# Autodesk Inventor assembly: House_Assembly
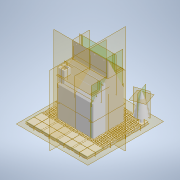
[picture p0: Inventor's stored thumbnail of the model, 180x180]
Saved by Autodesk Inventor 2022.4 (Build 264492010, 492A)
## iProperties
Created: 2025-02-20
Part Number: House_Assembly
Document SubType Name: Assembly
Designer: jan-m
Author: jan-m
## Documents named in this file (20)
- C:\School\Masterproef\3D Modellen\House_Assembly_Depth_Tracking.iam
- C:\School\Masterproef\3D Modellen\Tile.ipt
- C:\School\Masterproef\3D Modellen\Tile_Connector.ipt
- C:\School\Masterproef\3D Modellen\Wall.ipt
- C:\School\Masterproef\3D Modellen\Roof_Wall_Small_Left.ipt
- C:\School\Masterproef\3D Modellen\Roof_Wall_Small_Right.ipt
- C:\School\Masterproef\3D Modellen\Roof_Wall_Large_Left.ipt
- C:\School\Masterproef\3D Modellen\Roof_Wall_Large_Right.ipt
- C:\School\Masterproef\3D Modellen\Roof_Small.ipt
- C:\School\Masterproef\3D Modellen\Roof_Large.ipt
- C:\School\Masterproef\3D Modellen\Hanging_Wall.ipt
- C:\School\Masterproef\3D Modellen\1x1_Piece.ipt
- C:\School\Masterproef\3D Modellen\Tile_Cover.ipt
- C:\School\Masterproef\3D Modellen\Tree_Leaves.ipt
- C:\School\Masterproef\3D Modellen\Tree_Trunk.ipt
- C:\School\Masterproef\3D Modellen\Chimney.ipt
- C:\School\Masterproef\3D Modellen\Pin.ipt
- C:\School\Masterproef\3D Modellen\Rail_Clip_Left.ipt
- C:\School\Masterproef\3D Modellen\Rail_Clip_Right.ipt
- C:\School\Masterproef\3D Modellen\Roof_Pin_Clip.ipt
## Components (251 placed, 19 different names)
1. Wall:1 — Mate:10, Mate:11, Mate:12, Mate:40, Mate:46, Mate:59
2. Wall:2 — Mate:13, Mate:14, Mate:15, Mate:27, Mate:28, Mate:30, Mate:31, Mate:60, Mate:64, Mate:72
3. Wall:3 — Mate:19, Mate:20, Mate:21, Mate:37, Mate:42, Mate:58
4. Wall:4 — Mate:16, Mate:17, Mate:18, Mate:23, Mate:25, Mate:33, Mate:34, Mate:63, Mate:65
5. Roof_Wall_Small_Left:2 — Mate:23, Mate:25, Mate:65, Mate:80, Mate:81, Flush:6, Mate:102, Flush:12, Angle:1
6. Roof_Wall_Small_Right:2 — Mate:27, Mate:28, Mate:64, Mate:72, Mate:101, Mate:103, Flush:13, Angle:2
7. Roof_Wall_Large_Left:1 — Mate:30, Mate:31, Mate:60, Mate:106, Flush:16, Angle:5, Mate:107, Flush:17, Angle:6
8. Roof_Wall_Large_Right:1 — Mate:33, Mate:34, Mate:63, Mate:98, Mate:104, Flush:14, Angle:3, Mate:105, Flush:15, Angle:4
9. Roof_Small:1 — Mate:37, Mate:42, Mate:58, Mate:96, Mate:97, Mate:99, Mate:100
10. Roof_Large:1 — Mate:40, Mate:43, Mate:44, Mate:46, Mate:59, Flush:7
11. Hanging_Wall:1 — Mate:43, Mate:44, Flush:7
12. Tree_Leaves:1 — Mate:73, Mate:74
13. Tree_Trunk:1 — Mate:73, Mate:74, Mate:75, Mate:76, Mate:77
14. Chimney:1 — Mate:78, Mate:79, Mate:81, Flush:6
15. Pin:1 — Mate:78, Mate:79, Mate:80
16. Rail_Clip_Left:1 — Mate:96, Mate:97, Mate:98
17. Rail_Clip_Right:1 — Mate:99, Mate:100, Mate:101
18. Roof_Pin_Clip:1 — Mate:105, Flush:15, Angle:4
19. Roof_Pin_Clip:2 — Mate:106, Flush:16, Angle:5
20. Roof_Pin_Clip:3 — Mate:104, Flush:14, Angle:3
21. Roof_Pin_Clip:4 — Mate:102, Flush:12, Angle:1
22. Roof_Pin_Clip:5 — Mate:107, Flush:17, Angle:6
23. Roof_Pin_Clip:6 — Mate:103, Flush:13, Angle:2
24. Tile_Connector:2 — Mate:6, Mate:7
25. Tile:1 — Mate:2, Mate:5, Mate:6, Mate:7, Mate:16, Mate:91, Mate:92
26. Tile_Connector:1 — Mate:2, Mate:5
27. Tile_Connector:3
28. Tile:2 — Mate:10, Mate:12
29. Tile_Connector:4
30. Tile_Connector:5
31. Tile:3 — Mate:11
32. Tile_Connector:6
33. Tile_Connector:7
34. Tile:4 — Mate:13, Mate:75, Mate:76, Mate:77, Mate:94, Mate:95, Flush:11
35. Tile_Connector:8
36. Tile_Connector:9
37. Tile:5
38. Tile_Connector:10
39. Tile_Connector:11
40. Tile:6
41. Tile_Connector:12
42. Tile_Connector:13
43. Tile:7 — Mate:82, Flush:9
44. Tile_Connector:14
45. Tile_Connector:15
46. Tile:8 — Mate:15
47. Tile_Connector:16
48. Tile_Connector:17
49. Tile:9 — Mate:17, Mate:18, Mate:83, Mate:84, Flush:10, Mate:85, Mate:86
50. Tile_Connector:18
51. Tile_Connector:19
52. Tile:10 — Mate:19, Mate:21
53. Tile_Connector:20
54. Tile_Connector:21
55. Tile:11 — Mate:20
56. Tile_Connector:22
57. Tile_Connector:23
58. Tile:12 — Mate:14, Mate:88, Mate:89
59. Tile_Connector:24
60. Tile_Connector:25
61. Tile:13 — Mate:57, Mate:61, Mate:62
62. Tile_Connector:26
63. Tile_Connector:27
64. Tile:14
65. Tile_Connector:28
66. Tile_Connector:29
67. Tile:15
68. Tile_Connector:30
69. Tile_Connector:31
70. Tile:16
71. Tile_Connector:32
72. Tile_Cover:1 — Mate:57, Mate:61, Mate:62
73. Tile_Cover:2
74. Tile_Cover:3
75. Tile_Cover:4
76. 1x1_Piece:147 — Mate:83, Mate:84, Flush:10
77. 1x1_Piece:155
78. 1x1_Piece:156
79. 1x1_Piece:157 — Mate:87
80. 1x1_Piece:158
81. 1x1_Piece:159
82. 1x1_Piece:160
83. 1x1_Piece:161
84. 1x1_Piece:162
85. 1x1_Piece:163
86. 1x1_Piece:164
87. 1x1_Piece:165
88. 1x1_Piece:166
89. 1x1_Piece:167
90. 1x1_Piece:168
91. 1x1_Piece:169
92. 1x1_Piece:170
93. 1x1_Piece:171
94. 1x1_Piece:172
95. 1x1_Piece:173
96. 1x1_Piece:174
97. 1x1_Piece:175
98. 1x1_Piece:176
99. 1x1_Piece:177
100. 1x1_Piece:178
101. 1x1_Piece:179
102. 1x1_Piece:180
103. 1x1_Piece:181
104. 1x1_Piece:182
105. 1x1_Piece:183
106. 1x1_Piece:184
107. 1x1_Piece:185
108. 1x1_Piece:186
109. 1x1_Piece:187
110. 1x1_Piece:188
111. 1x1_Piece:189
112. 1x1_Piece:190
113. 1x1_Piece:191
114. 1x1_Piece:192
115. 1x1_Piece:193
116. 1x1_Piece:194
117. 1x1_Piece:195
118. 1x1_Piece:196
119. 1x1_Piece:197
120. 1x1_Piece:198
121. 1x1_Piece:199
122. 1x1_Piece:200
123. 1x1_Piece:201 — Mate:93
124. 1x1_Piece:202
125. 1x1_Piece:203
126. 1x1_Piece:204
127. 1x1_Piece:205
128. 1x1_Piece:206
129. 1x1_Piece:207
130. 1x1_Piece:208
131. 1x1_Piece:209
132. 1x1_Piece:210
133. 1x1_Piece:211
134. 1x1_Piece:212
135. 1x1_Piece:213
136. 1x1_Piece:146 — Mate:85, Mate:86, Mate:87
137. 1x1_Piece:214
138. 1x1_Piece:215
139. 1x1_Piece:216
140. 1x1_Piece:217
141. 1x1_Piece:218
142. 1x1_Piece:219
143. 1x1_Piece:220
144. 1x1_Piece:221
145. 1x1_Piece:222
146. 1x1_Piece:223
147. 1x1_Piece:224 — Mate:90
148. 1x1_Piece:151 — Mate:88, Mate:89, Mate:90
149. 1x1_Piece:225
150. 1x1_Piece:226
151. 1x1_Piece:227
152. 1x1_Piece:228
153. 1x1_Piece:229
154. 1x1_Piece:230
155. 1x1_Piece:231
156. 1x1_Piece:232
157. 1x1_Piece:233
158. 1x1_Piece:234
159. 1x1_Piece:235
160. 1x1_Piece:236
161. 1x1_Piece:237
162. 1x1_Piece:238
163. 1x1_Piece:239
164. 1x1_Piece:240
165. 1x1_Piece:241
166. 1x1_Piece:242
167. 1x1_Piece:243
168. 1x1_Piece:244
169. 1x1_Piece:245
170. 1x1_Piece:246
171. 1x1_Piece:247
172. 1x1_Piece:248
173. 1x1_Piece:249
174. 1x1_Piece:250
175. 1x1_Piece:251
176. 1x1_Piece:252
177. 1x1_Piece:253
178. 1x1_Piece:254
179. 1x1_Piece:255
180. 1x1_Piece:256
181. 1x1_Piece:257
182. 1x1_Piece:258
183. 1x1_Piece:259
184. 1x1_Piece:260
185. 1x1_Piece:261
186. 1x1_Piece:262
187. 1x1_Piece:263
188. 1x1_Piece:264
189. 1x1_Piece:265
190. 1x1_Piece:266
191. 1x1_Piece:267
192. 1x1_Piece:268
193. 1x1_Piece:269
194. 1x1_Piece:270
195. 1x1_Piece:271
196. 1x1_Piece:272
197. 1x1_Piece:273
198. 1x1_Piece:274
199. 1x1_Piece:275
200. 1x1_Piece:145 — Mate:91, Mate:92, Mate:93
201. 1x1_Piece:276
202. 1x1_Piece:277
203. 1x1_Piece:278
204. 1x1_Piece:279
205. 1x1_Piece:280
206. 1x1_Piece:281
207. 1x1_Piece:282
208. 1x1_Piece:283
209. 1x1_Piece:284
210. 1x1_Piece:285
211. 1x1_Piece:286
212. 1x1_Piece:287
213. 1x1_Piece:288
214. 1x1_Piece:289
215. 1x1_Piece:290
216. 1x1_Piece:291
217. 1x1_Piece:292
218. 1x1_Piece:293
219. 1x1_Piece:294
220. 1x1_Piece:295
221. 1x1_Piece:296
222. 1x1_Piece:297
223. 1x1_Piece:298
224. 1x1_Piece:299
225. 1x1_Piece:300
226. 1x1_Piece:301
227. 1x1_Piece:302
228. 1x1_Piece:303
229. 1x1_Piece:304
230. 1x1_Piece:305
231. 1x1_Piece:306
232. 1x1_Piece:307
233. 1x1_Piece:308
234. 1x1_Piece:309
235. 1x1_Piece:310
236. 1x1_Piece:311
237. 1x1_Piece:312
238. 1x1_Piece:313
239. 1x1_Piece:314
240. 1x1_Piece:315
241. 1x1_Piece:316
242. 1x1_Piece:317
243. 1x1_Piece:318
244. 1x1_Piece:319
245. 1x1_Piece:320
246. 1x1_Piece:321
247. 1x1_Piece:322
248. 1x1_Piece:148 — Mate:94, Mate:95, Flush:11
249. 1x1_Piece:323
250. 1x1_Piece:324
251. 1x1_Piece:325
## Component patterns: (16 elements, first: Tile_Connector:2 + Tile:1 + Tile_Connector:1), (4 elements, first: Tile_Cover:1), (60 elements, first: 1x1_Piece:147), (12 elements, first: 1x1_Piece:146), (52 elements, first: 1x1_Piece:151), (48 elements, first: 1x1_Piece:145), (4 elements, first: 1x1_Piece:148)
## Relationships (92: Mate 75, Flush 11, Angle 6)
- Mate:2: Tile:1 ↔ Tile_Connector:1
- Mate:5: Tile:1 ↔ Tile_Connector:1
- Mate:6: Tile_Connector:2 ↔ Tile:1
- Mate:7: Tile_Connector:2 ↔ Tile:1
- Mate:10: Wall:1 ↔ Tile:2
- Mate:11: Wall:1 ↔ Tile:3
- Mate:12: Wall:1 ↔ Tile:2
- Mate:13: Wall:2 ↔ Tile:4
- Mate:14: Wall:2 ↔ Tile:12
- Mate:15: Wall:2 ↔ Tile:8
- Mate:16: Wall:4 ↔ Tile:1
- Mate:17: Wall:4 ↔ Tile:9
- Mate:18: Wall:4 ↔ Tile:9
- Mate:19: Wall:3 ↔ Tile:10
- Mate:20: Wall:3 ↔ Tile:11
- Mate:21: Wall:3 ↔ Tile:10
- Mate:23: Wall:4 ↔ Roof_Wall_Small_Left:2
- Mate:25: Wall:4 ↔ Roof_Wall_Small_Left:2
- Mate:27: Wall:2 ↔ Roof_Wall_Small_Right:2
- Mate:28: Wall:2 ↔ Roof_Wall_Small_Right:2
- Mate:30: Wall:2 ↔ Roof_Wall_Large_Left:1
- Mate:31: Wall:2 ↔ Roof_Wall_Large_Left:1
- Mate:33: Wall:4 ↔ Roof_Wall_Large_Right:1
- Mate:34: Wall:4 ↔ Roof_Wall_Large_Right:1
- Mate:37: Wall:3 ↔ Roof_Small:1
- Mate:40: Wall:1 ↔ Roof_Large:1
- Mate:42: Wall:3 ↔ Roof_Small:1
- Mate:43: Roof_Large:1 ↔ Hanging_Wall:1
- Mate:44: Roof_Large:1 ↔ Hanging_Wall:1
- Mate:46: Wall:1 ↔ Roof_Large:1
- Mate:57: Tile:13 ↔ Tile_Cover:1
- Mate:58: Wall:3 ↔ Roof_Small:1
- Mate:59: Wall:1 ↔ Roof_Large:1
- Mate:60: Wall:2 ↔ Roof_Wall_Large_Left:1
- Mate:61: Tile:13 ↔ Tile_Cover:1
- Mate:62: Tile:13 ↔ Tile_Cover:1
- Mate:63: Wall:4 ↔ Roof_Wall_Large_Right:1
- Mate:64: Wall:2 ↔ Roof_Wall_Small_Right:2
- Mate:65: Wall:4 ↔ Roof_Wall_Small_Left:2
- Mate:72: Wall:2 ↔ Roof_Wall_Small_Right:2
- Mate:73: Tree_Leaves:1 ↔ Tree_Trunk:1
- Mate:74: Tree_Leaves:1 ↔ Tree_Trunk:1
- Mate:75: Tree_Trunk:1 ↔ Tile:4
- Mate:76: Tree_Trunk:1 ↔ Tile:4
- Mate:77: Tree_Trunk:1 ↔ Tile:4
- Mate:78: Chimney:1 ↔ Pin:1
- Mate:79: Chimney:1 ↔ Pin:1
- Mate:80: Roof_Wall_Small_Left:2 ↔ Pin:1
- Mate:81: Roof_Wall_Small_Left:2 ↔ Chimney:1
- Flush:6: Roof_Wall_Small_Left:2 ↔ Chimney:1
- Flush:7: Roof_Large:1 ↔ Hanging_Wall:1
- Mate:82: Tile:7
- Flush:9: Tile:7
- Mate:83: Tile:9 ↔ 1x1_Piece:147
- Mate:84: Tile:9 ↔ 1x1_Piece:147
- Flush:10: Tile:9 ↔ 1x1_Piece:147
- Mate:85: Tile:9 ↔ 1x1_Piece:146
- Mate:86: Tile:9 ↔ 1x1_Piece:146
- Mate:87: 1x1_Piece:157 ↔ 1x1_Piece:146
- Mate:88: Tile:12 ↔ 1x1_Piece:151
- Mate:89: Tile:12 ↔ 1x1_Piece:151
- Mate:90: 1x1_Piece:224 ↔ 1x1_Piece:151
- Mate:91: Tile:1 ↔ 1x1_Piece:145
- Mate:92: Tile:1 ↔ 1x1_Piece:145
- Mate:93: 1x1_Piece:201 ↔ 1x1_Piece:145
- Mate:94: Tile:4 ↔ 1x1_Piece:148
- Mate:95: Tile:4 ↔ 1x1_Piece:148
- Flush:11: Tile:4 ↔ 1x1_Piece:148
- Mate:96: Roof_Small:1 ↔ Rail_Clip_Left:1
- Mate:97: Roof_Small:1 ↔ Rail_Clip_Left:1
- Mate:98: Roof_Wall_Large_Right:1 ↔ Rail_Clip_Left:1
- Mate:99: Roof_Small:1 ↔ Rail_Clip_Right:1
- Mate:100: Roof_Small:1 ↔ Rail_Clip_Right:1
- Mate:101: Roof_Wall_Small_Right:2 ↔ Rail_Clip_Right:1
- Mate:102: Roof_Wall_Small_Left:2 ↔ Roof_Pin_Clip:4
- Flush:12: Roof_Wall_Small_Left:2 ↔ Roof_Pin_Clip:4
- Mate:103: Roof_Wall_Small_Right:2 ↔ Roof_Pin_Clip:6
- Flush:13: Roof_Wall_Small_Right:2 ↔ Roof_Pin_Clip:6
- Angle:1 (90 deg): Roof_Wall_Small_Left:2 ↔ Roof_Pin_Clip:4
- Angle:2 (90 deg): Roof_Wall_Small_Right:2 ↔ Roof_Pin_Clip:6
- Mate:104: Roof_Wall_Large_Right:1 ↔ Roof_Pin_Clip:3
- Flush:14: Roof_Wall_Large_Right:1 ↔ Roof_Pin_Clip:3
- Angle:3 (90 deg): Roof_Wall_Large_Right:1 ↔ Roof_Pin_Clip:3
- Mate:105: Roof_Wall_Large_Right:1 ↔ Roof_Pin_Clip:1
- Flush:15: Roof_Wall_Large_Right:1 ↔ Roof_Pin_Clip:1
- Angle:4 (90 deg): Roof_Wall_Large_Right:1 ↔ Roof_Pin_Clip:1
- Mate:106: Roof_Wall_Large_Left:1 ↔ Roof_Pin_Clip:2
- Flush:16: Roof_Wall_Large_Left:1 ↔ Roof_Pin_Clip:2
- Angle:5 (270 deg): Roof_Wall_Large_Left:1 ↔ Roof_Pin_Clip:2
- Mate:107: Roof_Wall_Large_Left:1 ↔ Roof_Pin_Clip:5
- Flush:17: Roof_Wall_Large_Left:1 ↔ Roof_Pin_Clip:5
- Angle:6 (90 deg): Roof_Wall_Large_Left:1 ↔ Roof_Pin_Clip:5
